# Autodesk Inventor assembly: 2019-7-4
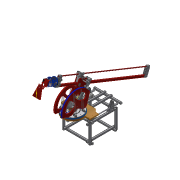
[picture p0: Inventor's stored thumbnail of the model, 180x180]
Saved by Autodesk Inventor 2019.4 (Build 234330000, 330)
## iProperties
Created: 2018-08-09
Part Number: 2019-7-4
Document SubType Name: Assembly
Designer: Owner
Mass: 3480.12 g
Surface Area: 17809.2 cm^2
Volume: 3279.54 cm^3
Density: 1.06116 g/cm^3
Author: Owner
## Documents named in this file (38)
- E:\ロボ研\キャチロボ\キャチロボ2019\CADdata\加工指示用\2019-7-4.iam
- E:\ロボ研\キャチロボ\キャチロボ2019\CADdata\アーム2019\2019HDarm\Slide_1.iam
- E:\ロボ研\キャチロボ\キャチロボ2019\CADdata\アーム2019\2019HDarm\Robot_Base.iam
- E:\ロボ研\キャチロボ\キャチロボ2019\CADdata\アーム2019\2019HDarm\Joint_1.iam
- E:\ロボ研\キャチロボ\キャチロボ2018\アーム\アーム01\回路ボックス.iam
- E:\ロボ研\キャチロボ\キャチロボ2019\CADdata\アーム2019\2019HDarm\Joint_3.iam
- E:\ロボ研\キャチロボ\キャチロボ2019\CADdata\アーム2019\2019HDarm\Pitch_B.ipt
- E:\ロボ研\キャチロボ\キャチロボ2019\CADdata\アーム2019\2019HDarm\p8-19flange.ipt
- E:\ロボ研\キャチロボ\キャチロボ2019\CADdata\アーム2019\2019HDarm\p8ALshaft.ipt
- E:\ロボ研\キャチロボ\キャチロボ2019\CADdata\アーム2019\KHK_SUMA120SUMA120On\AIS2019\SUMA1-20_SUMA1-20_On.iam
- E:\ロボ研\キャチロボ\キャチロボ2019\CADdata\アーム2019\2019HDarm\RS555PH_Geared_Motor.ipt
- E:\ロボ研\キャチロボ\キャチロボ2019\CADdata\アーム2019\PitchGears\PitchGears.iam
- E:\ロボ研\キャチロボ\キャチロボ2019\CADdata\アーム2019\PitchGears\PitchSquarePipe2.ipt
- E:\ロボ研\キャチロボ\キャチロボ2019\CADdata\アーム2019\PitchGears\RailWay.ipt
- E:\ロボ研\キャチロボ\キャチロボ2019\CADdata\アーム2019\SqPipeminin.ipt
- E:\ロボ研\キャチロボ\キャチロボ2019\CADdata\アーム2019\SqPipe92.ipt
- E:\ロボ研\キャチロボ\キャチロボ2019\CADdata\アーム2019\Tplate.ipt
- E:\ロボ研\キャチロボ\キャチロボ2019\CADdata\アーム2019\支え.ipt
- E:\ロボ研\キャチロボ\キャチロボ2019\CADdata\アーム2019\p9ALshaft.ipt
- E:\ロボ研\キャチロボ\キャチロボ2019\CADdata\アーム2019\Tplate_L.ipt
- E:\ロボ研\キャチロボ\キャチロボ2019\CADdata\アーム2019\p8-10_OilessFlange.ipt
- E:\ロボ研\キャチロボ\キャチロボ2019\CADdata\アーム2019\p8l65ALshaft.ipt
- E:\ロボ研\キャチロボ\キャチロボ2019\CADdata\アーム2019\RS555-71K_MotorsupportAL.ipt
- E:\ロボ研\キャチロボ\キャチロボ2019\CADdata\アーム2019\RS555-71K_MotorsupportPolica.ipt
- E:\ロボ研\キャチロボ\キャチロボ2019\CADdata\アーム2019\2019HDarm\p8ALshaftP.ipt
- E:\ロボ研\キャチロボ\キャチロボ2019\CADdata\アーム2019\2019HDarm\Key1.ipt
- E:\ロボ研\キャチロボ\キャチロボ2018\アーム\ポテンショメータB.ipt
- E:\ロボ研\キャチロボ\キャチロボ2018\アーム\アーム01\2axsisSensGear.ipt
- E:\ロボ研\キャチロボ\キャチロボ2019\CADdata\アーム2019\2019HDarm\FleLG.ipt
- E:\ロボ研\キャチロボ\キャチロボ2019\CADdata\plate2.ipt
- E:\ロボ研\キャチロボ\キャチロボ2019\CADdata\アーム2019\Wrist\Wrist.iam
- E:\ロボ研\キャチロボ\キャチロボ2019\CADdata\アーム2019\BaseSlider.iam
- E:\ロボ研\キャチロボ\キャチロボ2019\CADdata\アーム2019\BaseSlide_p10ALshaft.ipt
- E:\ロボ研\キャチロボ\キャチロボ2019\CADdata\アーム2019\BaseSupportSQpipe.ipt
- E:\ロボ研\キャチロボ\キャチロボ2019\CADdata\アーム2019\BaseSlideSTOPPERsq.ipt
- E:\ロボ研\キャチロボ\キャチロボ2019\CADdata\アーム2019\SlideHOLDsq.ipt
- E:\ロボ研\キャチロボ\キャチロボ2019\CADdata\アーム2019\BaseSlideSTOPPERsq2.ipt
- E:\ロボ研\キャチロボ\キャチロボ2018\アーム\アーム01\hand03\hand3.iam
## Components (60 placed, 37 different names)
1. Slide_1:1 [sub-assembly] — 設計用拘束, 設計用, 設計用3, リジッド:18, スライダ:5
2. Robot_Base:1 [sub-assembly] — フラッシュ:3, 設計用, 回転:11, スタート前, 設計用拘束4, 回転:12, 回転:13, リジッド:24
3. 回路ボックス:1 [sub-assembly] — スタート前, スタート後, 設計用拘束4, リジッド:22
4. Joint_1:1 [sub-assembly] — Fit, 挿入:16, 挿入:17, 角度:3, 挿入:22, 挿入:23, 挿入:43, 回転:3, 回転:11
5. Joint_3:1 [sub-assembly] — 設計用2, メイト:7, メイト:8, 正接:1, 挿入:38, 挿入:39, 回転:10, 挿入:52, スライダ:5
6. Pitch_B:1 — 設計用2, メイト:15, フラッシュ:7, メイト:16, 挿入:16, 挿入:17, 挿入:25, 挿入:26, 挿入:27, メイト:26, リジッド:6, リジッド:7, 挿入:47
7. p8ALshaft:1 — メイト:7, メイト:8, メイト:10, メイト:25, メイト:26, フラッシュ:11, メイト:27
8. SUMA1-20_SUMA1-20_On:1 [sub-assembly] — 挿入:3, メイト:15
9. RS555PH_Geared_Motor:1 — 挿入:3, フラッシュ:7, フラッシュ:10, リジッド:5
10. PitchGears:1 [sub-assembly] — メイト:10, Fit, メイト:16, 挿入:18, 挿入:19, 挿入:35, 挿入:49, 挿入:50
11. PitchGears:2 [sub-assembly] — 挿入:40, メイト:28, 回転:15
12. PitchSquarePipe2:1 — 挿入:18, 挿入:19, 挿入:52, フラッシュ:13, リジッド:16
13. PitchSquarePipe2:2 — 挿入:38, 挿入:39, 回転:15
14. RailWay:1 — 角度:3, 正接:1, メイト:25, 挿入:44, メイト:29
15. Tplate:1 — リジッド:1, リジッド:10, フラッシュ:11, メイト:29, 回転:14
16. 支え:1 — 挿入:25, 挿入:26, 挿入:27, 挿入:28, 挿入:29, 挿入:30, リジッド:1, 挿入:46
17. p9ALshaft:1 — 挿入:28
18. p9ALshaft:2 — 挿入:29
19. p9ALshaft:3 — 挿入:30
20. Tplate_L:1 — リジッド:11, 挿入:48, 回転:2, 回転:4, 回転:8, 回転:17, 回転:18
21. RailWay:2 — 回転:17, 回転:18
22. p8-10_OilessFlange:1 — 挿入:41
23. p8-10_OilessFlange:2 — 挿入:51
24. p8-19flange:1 — 挿入:35
25. p8-19flange:3 — 挿入:40, 挿入:41, メイト:27
26. Pitch_B:2 — 挿入:43, 回転:2, 回転:3, 回転:4, 挿入:51
27. p8l65ALshaft:1 — 挿入:44
28. SqPipe92:1 — リジッド:2
29. SqPipe92:2 — リジッド:3
30. RS555-71K_MotorsupportAL:1 — フラッシュ:10, リジッド:5, リジッド:6
31. RS555-71K_MotorsupportPolica:1 — リジッド:7
32. SqPipe92:3 — リジッド:10
33. SqPipe92:4 — リジッド:11
34. p8-10_OilessFlange:3 — 挿入:46
35. p8-10_OilessFlange:4 — 挿入:47
36. p8ALshaftP:1 — 挿入:48, フラッシュ:12, メイト:28, リジッド:12
37. Key1:1 — フラッシュ:12, 挿入:49, 挿入:50
38. Key1:2 — リジッド:12
39. 2axsisSensGear:1 — 正接:2
40. ポテンショメータB:2 — 回転:10
41. FleLG:1 — 回転:8, 正接:2
42. plate2:1 — フラッシュ:13, リジッド:16
43. Wrist:1 [sub-assembly] — リジッド:18, リジッド:31
44. BaseSlider:1 [sub-assembly] — 円柱状:1
45. BaseSlider:2 [sub-assembly] — リジッド:22, 円柱状:2
46. BaseSlide_p10ALshaft:1 — 円柱状:1, 平面:2, リジッド:26, リジッド:27
47. BaseSlide_p10ALshaft:2 — 円柱状:2, 平面:2, 回転:16
48. BaseSupportSQpipe:1 — 回転:12, 回転:13
49. BaseSupportSQpipe:2 — リジッド:24, リジッド:25
50. p8l65ALshaft:2 — 回転:14
51. BaseSlideSTOPPERsq:1 — リジッド:25, リジッド:27, スタート後, 回転:16
52. BaseSlideSTOPPERsq:2 — リジッド:26, リジッド:28, リジッド:29, リジッド:30
53. SlideHOLDsq:1 — リジッド:28
54. SlideHOLDsq:2 — リジッド:29
55. BaseSlideSTOPPERsq2:1 — リジッド:30
56. hand3:1 [sub-assembly] — リジッド:31
57. SqPipeminin:2 — 挿入:22, 挿入:23
58. SqPipeminin:3
59. SqPipeminin:4 — リジッド:2
60. SqPipeminin:5 — リジッド:3
## Component patterns: (4 elements, first: SqPipeminin:2)
## Relationships (100: Insert 27, WeldJoint 23, Mate 15, RevoluteJoint 14, Flush 10, Tangent 4, Angle 2, TranslationJoint 2, CylindricalJoint 2, PlanarJoint 1)
- [Flush]: Robot_Base:1
- [Flush]: Robot_Base:1
- フラッシュ:3 [Flush]: Robot_Base:1
- 設計用拘束 [Mate]: Slide_1:1
- 設計用 [Mate] (40 mm): Slide_1:1 ↔ Robot_Base:1
- 設計用3 [Flush]: Slide_1:1
- 設計用2 [Flush]: Joint_3:1 ↔ Pitch_B:1
- メイト:7 [Mate] (134 mm): Joint_3:1 ↔ p8ALshaft:1
- メイト:8 [Mate] (134 mm): Joint_3:1 ↔ p8ALshaft:1
- 挿入:3 [Insert] (-2 mm): SUMA1-20_SUMA1-20_On:1 ↔ RS555PH_Geared_Motor:1
- メイト:10 [Mate]: p8ALshaft:1 ↔ PitchGears:1
- Fit [Angle] (0 deg): Joint_1:1 ↔ PitchGears:1
- メイト:15 [Mate]: Pitch_B:1 ↔ SUMA1-20_SUMA1-20_On:1
- フラッシュ:7 [Flush]: Pitch_B:1 ↔ RS555PH_Geared_Motor:1
- メイト:16 [Mate]: Pitch_B:1 ↔ PitchGears:1
- 挿入:16 [Insert]: Joint_1:1 ↔ Pitch_B:1
- 挿入:17 [Insert]: Joint_1:1 ↔ Pitch_B:1
- 挿入:18 [Insert]: PitchGears:1 ↔ PitchSquarePipe2:1
- 挿入:19 [Insert]: PitchGears:1 ↔ PitchSquarePipe2:1
- 角度:3 [Angle] (90 deg): Joint_1:1 ↔ RailWay:1
- 正接:1 [Tangent]: Joint_3:1 ↔ RailWay:1
- メイト:25 [Mate]: p8ALshaft:1 ↔ RailWay:1
- 挿入:22 [Insert]: Joint_1:1 ↔ SqPipeminin:2
- 挿入:23 [Insert]: Joint_1:1 ↔ SqPipeminin:2
- 挿入:25 [Insert] (20 mm): Pitch_B:1 ↔ 支え:1
- 挿入:26 [Insert] (20 mm): Pitch_B:1 ↔ 支え:1
- 挿入:27 [Insert] (20 mm): Pitch_B:1 ↔ 支え:1
- 挿入:28 [Insert]: 支え:1 ↔ p9ALshaft:1
- 挿入:29 [Insert]: 支え:1 ↔ p9ALshaft:2
- 挿入:30 [Insert]: 支え:1 ↔ p9ALshaft:3
- リジッド:1 [WeldJoint]: Tplate:1 ↔ 支え:1
- 挿入:35 [Insert]: PitchGears:1 ↔ p8-19flange:1
- 挿入:38 [Insert]: Joint_3:1 ↔ PitchSquarePipe2:2
- 挿入:39 [Insert]: Joint_3:1 ↔ PitchSquarePipe2:2
- 挿入:40 [Insert]: PitchGears:2 ↔ p8-19flange:3
- メイト:26 [Mate]: Pitch_B:1 ↔ p8ALshaft:1
- 挿入:41 [Insert] (-0.5 mm): p8-10_OilessFlange:1 ↔ p8-19flange:3
- 挿入:43 [Insert]: Joint_1:1 ↔ Pitch_B:2
- 挿入:44 [Insert]: RailWay:1 ↔ p8l65ALshaft:1
- リジッド:2 [WeldJoint]: SqPipe92:1 ↔ SqPipeminin:4
- リジッド:3 [WeldJoint]: SqPipe92:2 ↔ SqPipeminin:5
- フラッシュ:10 [Flush]: RS555PH_Geared_Motor:1 ↔ RS555-71K_MotorsupportAL:1
- リジッド:5 [WeldJoint]: RS555PH_Geared_Motor:1 ↔ RS555-71K_MotorsupportAL:1
- リジッド:6 [WeldJoint]: Pitch_B:1 ↔ RS555-71K_MotorsupportAL:1
- リジッド:7 [WeldJoint]: Pitch_B:1 ↔ RS555-71K_MotorsupportPolica:1
- リジッド:10 [WeldJoint]: Tplate:1 ↔ SqPipe92:3
- リジッド:11 [WeldJoint]: Tplate_L:1 ↔ SqPipe92:4
- 挿入:46 [Insert]: 支え:1 ↔ p8-10_OilessFlange:3
- 挿入:47 [Insert]: Pitch_B:1 ↔ p8-10_OilessFlange:4
- フラッシュ:11 [Flush]: p8ALshaft:1 ↔ Tplate:1
- 挿入:48 [Insert]: Tplate_L:1 ↔ p8ALshaftP:1
- フラッシュ:12 [Flush]: p8ALshaftP:1 ↔ Key1:1
- 挿入:49 [Insert]: PitchGears:1 ↔ Key1:1
- 挿入:50 [Insert]: PitchGears:1 ↔ Key1:1
- 回転:2 [RevoluteJoint]: Tplate_L:1 ↔ Pitch_B:2
- 回転:3 [RevoluteJoint]: Joint_1:1 ↔ Pitch_B:2
- 回転:4 [RevoluteJoint]: Tplate_L:1 ↔ Pitch_B:2
- メイト:27 [Mate]: p8ALshaft:1 ↔ p8-19flange:3
- メイト:28 [Mate]: PitchGears:2 ↔ p8ALshaftP:1
- リジッド:12 [WeldJoint]: p8ALshaftP:1 ↔ Key1:2
- [RevoluteJoint] (-1 mm): 2axsisSensGear:1 ↔ ポテンショメータB:2
- 回転:8 [RevoluteJoint]: Tplate_L:1 ↔ FleLG:1
- 正接:2 [Tangent]: 2axsisSensGear:1 ↔ FleLG:1
- 回転:10 [RevoluteJoint]: Joint_3:1 ↔ ポテンショメータB:2
- 挿入:51 [Insert]: p8-10_OilessFlange:2 ↔ Pitch_B:2
- 回転:11 [RevoluteJoint]: Robot_Base:1 ↔ Joint_1:1
- 挿入:52 [Insert]: Joint_3:1 ↔ PitchSquarePipe2:1
- メイト:29 [Mate]: RailWay:1 ↔ Tplate:1
- フラッシュ:13 [Flush]: PitchSquarePipe2:1 ↔ plate2:1
- リジッド:16 [WeldJoint]: PitchSquarePipe2:1 ↔ plate2:1
- リジッド:18 [WeldJoint]: Slide_1:1 ↔ Wrist:1
- スタート前 [Mate] (8 mm): Robot_Base:1 ↔ 回路ボックス:1
- スタート後 [Mate] (50 mm): 回路ボックス:1 ↔ BaseSlideSTOPPERsq:1
- 設計用拘束4 [TranslationJoint] (35 mm): Robot_Base:1 ↔ 回路ボックス:1
- [Mate]: 回路ボックス:1 ↔ BaseSlider:1
- [Tangent]: 回路ボックス:1 ↔ BaseSlider:1
- [Tangent]: 回路ボックス:1 ↔ BaseSlider:1
- [WeldJoint]: 回路ボックス:1 ↔ BaseSlider:1
- [WeldJoint]: 回路ボックス:1 ↔ BaseSlider:1
- [WeldJoint]: 回路ボックス:1 ↔ BaseSlider:1
- リジッド:22 [WeldJoint]: 回路ボックス:1 ↔ BaseSlider:2
- 円柱状:1 [CylindricalJoint]: BaseSlider:1 ↔ BaseSlide_p10ALshaft:1
- 円柱状:2 [CylindricalJoint]: BaseSlider:2 ↔ BaseSlide_p10ALshaft:2
- 平面:2 [PlanarJoint]: BaseSlide_p10ALshaft:1 ↔ BaseSlide_p10ALshaft:2
- 回転:12 [RevoluteJoint]: Robot_Base:1 ↔ BaseSupportSQpipe:1
- 回転:13 [RevoluteJoint]: Robot_Base:1 ↔ BaseSupportSQpipe:1
- リジッド:24 [WeldJoint]: Robot_Base:1 ↔ BaseSupportSQpipe:2
- 回転:14 [RevoluteJoint] (-3 mm): Tplate:1 ↔ p8l65ALshaft:2
- 回転:15 [RevoluteJoint]: PitchGears:2 ↔ PitchSquarePipe2:2
- リジッド:25 [WeldJoint]: BaseSupportSQpipe:2 ↔ BaseSlideSTOPPERsq:1
- リジッド:26 [WeldJoint]: BaseSlide_p10ALshaft:1 ↔ BaseSlideSTOPPERsq:2
- リジッド:27 [WeldJoint]: BaseSlide_p10ALshaft:1 ↔ BaseSlideSTOPPERsq:1
- リジッド:28 [WeldJoint]: BaseSlideSTOPPERsq:2 ↔ SlideHOLDsq:1
- リジッド:29 [WeldJoint]: BaseSlideSTOPPERsq:2 ↔ SlideHOLDsq:2
- リジッド:30 [WeldJoint] (-18 mm): BaseSlideSTOPPERsq:2 ↔ BaseSlideSTOPPERsq2:1
- 回転:16 [RevoluteJoint]: BaseSlide_p10ALshaft:2 ↔ BaseSlideSTOPPERsq:1
- 回転:17 [RevoluteJoint]: Tplate_L:1 ↔ RailWay:2
- 回転:18 [RevoluteJoint]: Tplate_L:1 ↔ RailWay:2
- リジッド:31 [WeldJoint]: Wrist:1 ↔ hand3:1
- スライダ:5 [TranslationJoint]: Slide_1:1 ↔ Joint_3:1
